# Autodesk Inventor assembly: haha
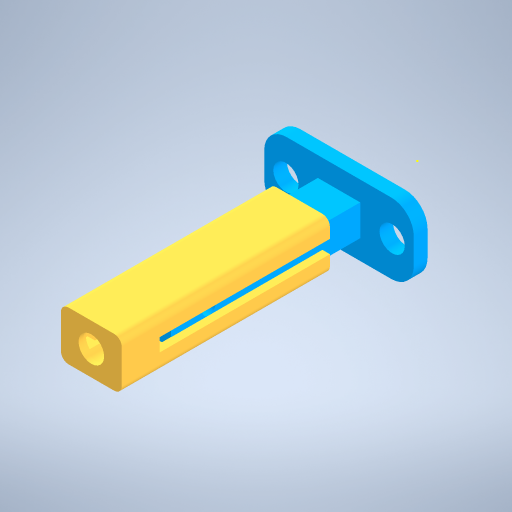
[picture p0: Inventor's stored thumbnail of the model, 512x512]
Saved by Autodesk Inventor 2024 (Build 280153000, 153)
## iProperties
Created: 2024-02-10
Part Number: haha
Document SubType Name: Assembly
Designer: MSI USER
Author: MSI USER
## Documents named in this file (3)
- C:\Users\MSI USER\Downloads\haha.iam
- C:\Users\MSI USER\Downloads\trughep_small.ipt
- C:\Users\MSI USER\Downloads\trughep2_small.ipt
## Components (2 placed, 2 different names)
1. trughep_small:1 — Mate:1, Mate:2, Mate:3
2. trughep2_small:1 — Mate:2, Mate:3
## Relationships (3: Mate 3)
- Mate:1: trughep_small:1
- Mate:2 (0.4 mm): trughep_small:1 ↔ trughep2_small:1
- Mate:3 (10 mm): trughep_small:1 ↔ trughep2_small:1
